# Autodesk Inventor assembly: Turtle3
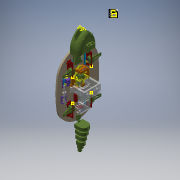
[picture p0: Inventor's stored thumbnail of the model, 180x180]
Saved by Autodesk Inventor 2018 (Build 220112000, 112)
## iProperties
Created: 2018-05-19
Part Number: Turtle3
Document SubType Name: Assembly
Designer: reide
Author: reide
## Documents named in this file (69)
- C:\Users\reide\OneDrive\Documents\Inventor\TSA\2018\Animatronics\Tortoise\Turtle3.iam
- C:\Users\reide\OneDrive\Documents\Inventor\TSA\2018\Animatronics\Tortoise\Frame\Frame - Copy.ipt
- C:\Users\reide\OneDrive\Documents\Inventor\TSA\2018\Animatronics\Tortoise\Rack.ipt
- C:\Users\reide\OneDrive\Documents\Inventor\TSA\2018\Animatronics\Tortoise\arms\Supporter.ipt
- C:\Users\reide\OneDrive\Documents\Inventor\TSA\2018\Animatronics\Tortoise\arms\GuideArm.ipt
- C:\Users\reide\OneDrive\Documents\Inventor\TSA\2018\Animatronics\Tortoise\arms\GuideArmConnector.ipt
- C:\Users\reide\OneDrive\Documents\Inventor\TSA\2018\Animatronics\Tortoise\arms\GuideArmConnectorLimitSwitch.ipt
- C:\Users\reide\OneDrive\Documents\Inventor\TSA\2018\Animatronics\Tortoise\arms\newShoulder_MIR.ipt
- C:\Users\reide\OneDrive\Documents\Inventor\TSA\2018\Animatronics\Tortoise\arms\straightBar_MIR.ipt
- C:\Users\reide\OneDrive\Documents\Inventor\TSA\2018\Animatronics\Tortoise\arms\AngleArm_MIR.ipt
- C:\Users\reide\OneDrive\Documents\Inventor\TSA\2018\Animatronics\Tortoise\arms\bottomARM_MIR.ipt
- C:\Users\reide\OneDrive\Documents\Inventor\TSA\2018\Animatronics\Tortoise\Mock Parts\servo (2)_MIR.ipt
- C:\Users\reide\OneDrive\Documents\Inventor\TSA\2018\Animatronics\Tortoise\Pinion final_MIR.ipt
- C:\Users\reide\OneDrive\Documents\Inventor\TSA\2018\Animatronics\Tortoise\arms\newShoulder.ipt
- C:\Users\reide\OneDrive\Documents\Inventor\TSA\2018\Animatronics\Tortoise\arms\straightBar.ipt
- C:\Users\reide\OneDrive\Documents\Inventor\TSA\2018\Animatronics\Tortoise\arms\AngleArm.ipt
- C:\Users\reide\OneDrive\Documents\Inventor\TSA\2018\Animatronics\Tortoise\arms\bottomARM.ipt
- C:\Users\reide\OneDrive\Documents\Inventor\TSA\2018\Animatronics\Tortoise\Mock Parts\servo (2).ipt
- C:\Users\reide\OneDrive\Documents\Inventor\TSA\2018\Animatronics\Tortoise\Pinion final.ipt
- C:\Users\reide\OneDrive\Documents\Inventor\TSA\2018\Animatronics\Tortoise\Head\HeadBasePt1.iam
- C:\Users\reide\OneDrive\Documents\Inventor\TSA\2018\Animatronics\Tortoise\Head\HeadBasePt2.iam
- C:\Users\reide\OneDrive\Documents\Inventor\TSA\2018\Animatronics\Tortoise\Head\HeadBottom1.ipt
- C:\Users\reide\OneDrive\Documents\Inventor\TSA\2018\Animatronics\Tortoise\Head\SyringeAttachment.ipt
- C:\Users\reide\OneDrive\Documents\Inventor\TSA\2018\Animatronics\Tortoise\Syringe3mL\SyringeBody.ipt
- C:\Users\reide\OneDrive\Documents\Inventor\TSA\2018\Animatronics\Tortoise\Syringe3mL\SyringEnd.ipt
- C:\Users\reide\OneDrive\Documents\Inventor\TSA\2018\Animatronics\Tortoise\Head\HeadBottom.ipt
- C:\Users\reide\OneDrive\Documents\Inventor\TSA\2018\Animatronics\Tortoise\Head\HeadLever.ipt
- C:\Users\reide\OneDrive\Documents\Inventor\TSA\2018\Animatronics\Tortoise\Head\FlexHinge.ipt
- C:\Users\reide\OneDrive\Documents\Inventor\TSA\2018\Animatronics\Tortoise\Head\HeadTop.ipt
- C:\Users\reide\OneDrive\Documents\Inventor\TSA\2018\Animatronics\Tortoise\Head\Face.ipt
- C:\Users\reide\OneDrive\Documents\Inventor\TSA\2018\Animatronics\Tortoise\Head\Eyes.ipt
- C:\Users\reide\OneDrive\Documents\Inventor\TSA\2018\Animatronics\Tortoise\Head\SensorMount.ipt
- C:\Users\reide\OneDrive\Documents\Inventor\TSA\2018\Animatronics\Tortoise\Wheels\smallergear.ipt
- C:\Users\reide\OneDrive\Documents\Inventor\TSA\2018\Animatronics\Tortoise\Clamps\SteerServoClamp.ipt
- C:\Users\reide\OneDrive\Documents\Inventor\TSA\2018\Animatronics\Tortoise\Wheels\steer_servo_mount1.ipt
- C:\Users\reide\OneDrive\Documents\Inventor\TSA\2018\Animatronics\Tortoise\Wheels\steer_servo_mount2.ipt
- C:\Users\reide\OneDrive\Documents\Inventor\TSA\2018\Animatronics\Tortoise\Wheels\wheelframe2NEW.ipt
- C:\Users\reide\OneDrive\Documents\Inventor\TSA\2018\Animatronics\Tortoise\Wheels\wheelframe.ipt
- C:\Users\reide\OneDrive\Documents\Inventor\TSA\2018\Animatronics\Tortoise\Wheels\wheel gear.ipt
- C:\Users\reide\OneDrive\Documents\Inventor\TSA\2018\Animatronics\Tortoise\Wheels\correct_wheel.ipt
- C:\Users\reide\OneDrive\Documents\Inventor\TSA\2018\Animatronics\Tortoise\Wheels\holder_gear_mount1.ipt
- C:\Users\reide\OneDrive\Documents\Inventor\TSA\2018\Animatronics\Tortoise\Wheels\holder_gear_mount2.ipt
- C:\Users\reide\OneDrive\Documents\Inventor\TSA\2018\Animatronics\Tortoise\Wheels\BackWheelMount.ipt
- C:\Users\reide\OneDrive\Documents\Inventor\TSA\2018\Animatronics\Tortoise\Wheels\BackWheelServoClasp.ipt
- C:\Users\reide\OneDrive\Documents\Inventor\TSA\2018\Animatronics\Tortoise\Wheels\Backwheel.ipt
- C:\Users\reide\OneDrive\Documents\Inventor\TSA\2018\Animatronics\Tortoise\Tail\Tail_Servo_Mount.ipt
- C:\Users\reide\OneDrive\Documents\Inventor\TSA\2018\Animatronics\Tortoise\Tail\Tail_Mount.ipt
- C:\Users\reide\OneDrive\Documents\Inventor\TSA\2018\Animatronics\Tortoise\Tail\Tail3.ipt
- C:\Users\reide\OneDrive\Documents\Inventor\TSA\2018\Animatronics\Tortoise\Tail\Tail4.ipt
- C:\Users\reide\OneDrive\Documents\Inventor\TSA\2018\Animatronics\Tortoise\Tail\Tail5.ipt
- C:\Users\reide\OneDrive\Documents\Inventor\TSA\2018\Animatronics\Tortoise\Tail\Tail6.ipt
- C:\Users\reide\OneDrive\Documents\Inventor\TSA\2018\Animatronics\Tortoise\Frame\TablePt1.ipt
- C:\Users\reide\OneDrive\Documents\Inventor\TSA\2018\Animatronics\Tortoise\Frame\TablePt2.ipt
- C:\Users\reide\OneDrive\Documents\Inventor\TSA\2018\Animatronics\Tortoise\Frame\TableLeg.ipt
- C:\Users\reide\OneDrive\Documents\Inventor\TSA\2018\Animatronics\Tortoise\Frame\ButtonMountLegs.ipt
- C:\Users\reide\OneDrive\Documents\Inventor\TSA\2018\Animatronics\Tortoise\Frame\ButtonMountCarrier.ipt
- C:\Users\reide\OneDrive\Documents\Inventor\TSA\2018\Animatronics\Tortoise\Frame\ButtonMount.ipt
- C:\Users\reide\OneDrive\Documents\Inventor\TSA\2018\Animatronics\Tortoise\Head\HeadOpenRack.ipt
- C:\Users\reide\OneDrive\Documents\Inventor\TSA\2018\Animatronics\Tortoise\Frame\SyringeMotorBase_MIR.ipt
- C:\Users\reide\OneDrive\Documents\Inventor\TSA\2018\Animatronics\Tortoise\Clamps\SyringeServoBaseClamp_MIR.ipt
- C:\Users\reide\OneDrive\Documents\Inventor\TSA\2018\Animatronics\Tortoise\Frame\BaseSyringeRackWall.ipt
- C:\Users\reide\OneDrive\Documents\Inventor\TSA\2018\Animatronics\Tortoise\Clamps\SyringeBaseSlotters.ipt
- C:\Users\reide\OneDrive\Documents\Inventor\TSA\2018\Animatronics\Tortoise\Head\SyringeHeadLeverAttachment.ipt
- C:\Users\reide\OneDrive\Documents\Inventor\TSA\2018\Animatronics\Tortoise\Head\LeverArm.ipt
- C:\Users\reide\OneDrive\Documents\Inventor\TSA\2018\Animatronics\Tortoise\Head\HeadLeverAssemblyAttacher.ipt
- C:\Users\reide\OneDrive\Documents\Inventor\TSA\2018\Animatronics\Tortoise\Frame\ThumbScrew.ipt
- C:\Users\reide\OneDrive\Documents\Inventor\TSA\2018\Animatronics\Tortoise\Clamps\SyringeServoClamp.ipt
- C:\Users\reide\OneDrive\Documents\Inventor\TSA\2018\Animatronics\Tortoise\Frame\ButtonLockerV2.ipt
- C:\Users\reide\OneDrive\Documents\Inventor\TSA\2018\Animatronics\Tortoise\Frame\FrameRim.ipt
## Components (131 placed, 68 different names)
1. Frame - Copy:1 — Mate:17, Mate:18, Mate:19, Mate:20, Mate:21, Mate:22, Mate:23, Mate:24, Mate:25, Mate:26, Mate:27, Mate:28, Mate:29, Mate:30, Mate:31, Mate:32, Mate:33, Mate:34, Mate:35, Mate:36, Mate:37, Mate:38, Mate:39, Mate:40, Mate:41, Mate:88, Mate:89, Mate:90, Mate:144, Mate:145, Mate:157, Mate:158, Mate:161, Mate:162, Mate:167, Mate:168, Mate:169, Mate:175, Mate:176, Mate:177, Mate:178, Mate:179, Mate:180, Mate:181, Mate:182, Mate:183, Mate:184, Mate:185, Mate:186, Mate:187, Mate:203, Mate:204, Mate:205, Mate:206, Mate:207, Mate:208, Mate:209, Mate:210, Mate:241, Mate:242, Mate:243, Mate:244, Mate:245, Flush:106, Mate:246, Mate:247, Flush:107, Mate:248, Mate:249, Mate:250, Mate:254, Flush:111, Mate:295, Mate:296, Flush:114
2. Rack:1 — Flush:6, Flush:25, Flush:26, Flush:27, Mate:22, Mate:23
3. Supporter:1 — Flush:5, Flush:6, Mate:17, Mate:18, Mate:19, Mate:51, Angle:9
4. GuideArm:1 — Mate:52
5. GuideArmConnector:1 — Mate:21
6. GuideArmConnectorLimitSwitch:1 — Flush:5, Mate:20
7. Rack:2 — Mate:28, Mate:29
8. Supporter:2 — Flush:25, Mate:24, Mate:25, Mate:80
9. GuideArm:2 — Mate:81
10. GuideArmConnector:2 — Mate:27
11. GuideArmConnectorLimitSwitch:2 — Mate:26
12. Rack:3 — Mate:40, Mate:41
13. Supporter:3 — Flush:27, Mate:36, Mate:37, Mate:85
14. GuideArm:3 — Mate:84
15. GuideArmConnector:3 — Mate:38
16. GuideArmConnectorLimitSwitch:3 — Mate:39
17. Rack:4 — Mate:34, Mate:35
18. Supporter:4 — Flush:26, Mate:30, Mate:31, Mate:83
19. GuideArm:4 — Mate:82
20. GuideArmConnector:4 — Mate:32
21. GuideArmConnectorLimitSwitch:4 — Mate:33
22. newShoulder_MIR:1 — Mate:50, Mate:51, Mate:52
23. straightBar_MIR:1
24. AngleArm_MIR:1 — Angle:8
25. bottomARM_MIR:1
26. servo (2)_MIR:1 — Mate:50
27. Pinion final_MIR:1
28. newShoulder_MIR:2 — Mate:84, Mate:85
29. straightBar_MIR:2
30. AngleArm_MIR:2
31. bottomARM_MIR:2
32. servo (2)_MIR:2
33. Pinion final_MIR:2
34. newShoulder:1 — Mate:70, Mate:80, Mate:81
35. straightBar:1
36. AngleArm:1
37. bottomARM:1
38. servo (2):1 — Mate:70
39. Pinion final:1
40. newShoulder:2 — Mate:82, Mate:83
41. straightBar:2
42. AngleArm:2
43. bottomARM:2
44. servo (2):2
45. Pinion final:2
46. HeadBasePt1:1 [sub-assembly] — Mate:86, Flush:48, Mate:87, Mate:89, Mate:90, Mate:127, Mate:128, Angle:2, Angle:3
47. HeadBasePt2:1 [sub-assembly] — Mate:86, Flush:48, Mate:87, Mate:88
48. servo (2):3 — Mate:131, Mate:132
49. HeadBottom1:1 — Mate:107, Mate:127, Mate:128, Angle:2, Flush:108, Mate:271, Mate:272
50. SyringeAttachment:1 — Angle:1
51. SyringeAttachment:2
52. servo (2):4 — Mate:129, Mate:130
53. SyringeBody:1 — Angle:1, Mate:107
54. SyringEnd:1 — Mate:261, Mate:262
55. HeadLever:1 — Mate:263, Mate:267, Mate:270, Mate:282, Mate:283, Mate:285
56. FlexHinge:1 — Mate:274, Mate:276, Angle:10
57. HeadTop:1 — Mate:119, Mate:263, Flush:110, Mate:284, Mate:285
58. Face:1 — Mate:119, Mate:120, Mate:298, Mate:299
59. FlexHinge:2 — Mate:273, Mate:275, Angle:9
60. Eyes:1 — Mate:120
61. Eyes:2
62. Pinion final:3 — Mate:129, Mate:130
63. Pinion final:4 — Mate:131, Mate:132
64. servo (2):5 — Mate:136, Mate:137, Mate:138, Mate:139, Mate:140
65. smallergear:1 — Mate:139, Mate:140
66. SteerServoClamp:1 — Mate:141, Mate:142, Mate:143
67. steer_servo_mount1:1 — Mate:134, Mate:135, Flush:54, Flush:55, Flush:56, Flush:57, Mate:136, Mate:137, Mate:138, Mate:141, Mate:142, Mate:143, Angle:3, Angle:4
68. steer_servo_mount2:1 — Mate:134, Flush:56, Flush:57, Mate:144, Mate:145
69. steer_servo_mount2:2 — Mate:135, Flush:54, Flush:55, Angle:5
70. wheelframe2NEW:1 — Mate:158
71. wheelframe:1 — Mate:153, Mate:154, Mate:155, Mate:157
72. wheel gear:1 — Flush:58, Mate:156
73. correct_wheel:1 — Flush:58
74. servo (2):7 — Mate:153, Mate:154, Mate:155, Mate:156
75. smallergear:2 — Flush:64, Mate:160
76. holder_gear_mount1:1 — Mate:159, Flush:60, Flush:61, Flush:62, Flush:63, Flush:64, Mate:160, Angle:4
77. holder_gear_mount2:1 — Flush:59, Mate:159, Flush:60, Flush:61, Mate:161, Mate:162
78. holder_gear_mount2:2 — Flush:59, Flush:62, Flush:63, Angle:6
79. smallergear:3
80. holder_gear_mount1:2
81. holder_gear_mount2:3 — Flush:77, Mate:167, Mate:169, Angle:6
82. holder_gear_mount2:4
83. smallergear:4
84. holder_gear_mount1:3
85. holder_gear_mount2:5 — Flush:77, Mate:168, Angle:5
86. holder_gear_mount2:6 — Angle:7
87. BackWheelMount:1 — Mate:178, Mate:179, Mate:180
88. BackWheelServoClasp:1 — Flush:79, Mate:175, Mate:176, Mate:177
89. Backwheel:1 — Mate:181
90. Tail_Servo_Mount:1 — Mate:182, Mate:183, Mate:184
91. servo (2):8 — Flush:79
92. servo (2):9
93. Tail_Mount:1 — Mate:185, Mate:186, Mate:187, Mate:188, Mate:189
94. Tail3:1 — Mate:188, Mate:189, Mate:190, Mate:191
95. Tail4:1 — Mate:190, Mate:191, Mate:192, Mate:193
96. Tail5:1 — Mate:192, Mate:193, Mate:194, Mate:195
97. Tail6:1 — Mate:194, Mate:195
98. TablePt1:1 — Mate:196, Flush:80, Flush:86, Mate:199, Mate:201, Mate:202, Flush:88, Mate:203
99. TablePt2:1 — Mate:196, Flush:80, Mate:198, Flush:81, Flush:82, Flush:87, Mate:200, Flush:88, Angle:7, Mate:286, Flush:112, Flush:113
100. TableLeg:1 — Mate:198, Flush:81, Flush:82, Flush:85
101. TableLeg:2 — Flush:83, Mate:201, Mate:202, Mate:204
102. TableLeg:3 — Flush:83, Flush:84, Flush:87, Mate:200
103. TableLeg:4 — Flush:84, Flush:85, Flush:86, Mate:199
104. ButtonMountLegs:1 — Mate:205, Mate:206, Mate:207, Mate:211, Angle:12
105. ButtonMountLegs:2 — Mate:208, Mate:209, Mate:210, Flush:90, Flush:91
106. ButtonMount:1 — Flush:90, Flush:91, Mate:211, Mate:287, Mate:288, Angle:11
107. SyringeBody:3 — Mate:245, Mate:297
108. SyringeAttachment:5 — Mate:247
109. SyringeAttachment:6 — Mate:246
110. servo (2)_MIR:4 — Mate:239, Flush:105, Mate:240
111. Pinion final:6
112. SyringeMotorBase_MIR:1 — Flush:103, Flush:104, Mate:238, Mate:239, Flush:105, Mate:240, Mate:241, Mate:242, Mate:243, Mate:244
113. SyringeServoBaseClamp_MIR:1 — Flush:103, Flush:104, Mate:238
114. BaseSyringeRackWall:1 — Flush:106, Mate:253, Mate:295, Mate:296
115. SyringeBaseSlotters:1 — Flush:107
116. SyringeBaseSlotters:2 — Mate:248, Mate:249, Mate:250
117. HeadOpenRack:3 — Mate:253, Mate:254
118. SyringEnd:4 — Mate:297
119. SyringeHeadLeverAttachment:1 — Mate:261, Mate:262, Angle:8, Mate:265, Mate:266, Mate:268, Mate:269
120. LeverArm:2 — Mate:265, Mate:266, Mate:267
121. LeverArm:3 — Mate:268, Mate:269, Mate:270
122. HeadLeverAssemblyAttacher:1 — Mate:277, Mate:278, Mate:279, Flush:109, Mate:282, Mate:283
123. HeadBottom:2 — Flush:108, Mate:271, Mate:272, Mate:273, Mate:274, Mate:275, Mate:276, Angle:10, Mate:277, Mate:278, Mate:279, Mate:280, Mate:281, Flush:110, Mate:284, Angle:14
124. HeadLeverAssemblyAttacher:2 — Mate:280, Flush:109, Mate:281
125. ThumbScrew:1 — Flush:111
126. SyringeServoClamp:1 — Mate:286, Flush:112, Flush:113
127. ButtonMountCarrier:2 — Mate:287, Mate:288, Angle:11, Mate:292, Angle:13
128. ButtonLockerV2:2 — Mate:292, Angle:12
129. ButtonLockerV2:3 — Angle:13
130. FrameRim:1 — Flush:114
131. SensorMount:2 — Mate:298, Angle:14, Mate:299
## Relationships (361: Mate 249, Flush 98, Angle 14)
- [Flush]: Rack:1 ↔ Supporter:1
- [Mate]: GuideArm:1 ↔ GuideArmConnector:1
- [Mate]: GuideArm:1 ↔ GuideArmConnector:1
- [Flush]: GuideArm:1 ↔ GuideArmConnector:1
- [Flush]: GuideArmConnector:1 ↔ GuideArmConnectorLimitSwitch:1
- [Mate]: GuideArm:1 ↔ GuideArmConnectorLimitSwitch:1
- [Flush]: GuideArm:1 ↔ GuideArmConnectorLimitSwitch:1
- [Mate]: GuideArm:1 ↔ GuideArmConnectorLimitSwitch:1
- Flush:5: Supporter:1 ↔ GuideArmConnectorLimitSwitch:1
- Flush:6: Rack:1 ↔ Supporter:1
- [Flush]: Rack:2 ↔ Supporter:2
- [Mate]: GuideArm:2 ↔ GuideArmConnector:2
- [Mate]: GuideArm:2 ↔ GuideArmConnector:2
- [Flush]: GuideArm:2 ↔ GuideArmConnector:2
- [Flush]: GuideArmConnector:2 ↔ GuideArmConnectorLimitSwitch:2
- [Mate]: GuideArm:2 ↔ GuideArmConnectorLimitSwitch:2
- [Flush]: GuideArm:2 ↔ GuideArmConnectorLimitSwitch:2
- [Mate]: GuideArm:2 ↔ GuideArmConnectorLimitSwitch:2
- [Flush]: Supporter:2 ↔ GuideArmConnectorLimitSwitch:2
- [Flush]: Rack:2 ↔ Supporter:2
- [Flush]: Rack:3 ↔ Supporter:3
- [Mate]: GuideArm:3 ↔ GuideArmConnector:3
- [Mate]: GuideArm:3 ↔ GuideArmConnector:3
- [Flush]: GuideArm:3 ↔ GuideArmConnector:3
- [Flush]: GuideArmConnector:3 ↔ GuideArmConnectorLimitSwitch:3
- [Mate]: GuideArm:3 ↔ GuideArmConnectorLimitSwitch:3
- [Flush]: GuideArm:3 ↔ GuideArmConnectorLimitSwitch:3
- [Mate]: GuideArm:3 ↔ GuideArmConnectorLimitSwitch:3
- [Flush]: Supporter:3 ↔ GuideArmConnectorLimitSwitch:3
- [Flush]: Rack:3 ↔ Supporter:3
- [Flush]: Rack:4 ↔ Supporter:4
- [Mate]: GuideArm:4 ↔ GuideArmConnector:4
- [Mate]: GuideArm:4 ↔ GuideArmConnector:4
- [Flush]: GuideArm:4 ↔ GuideArmConnector:4
- [Flush]: GuideArmConnector:4 ↔ GuideArmConnectorLimitSwitch:4
- [Mate]: GuideArm:4 ↔ GuideArmConnectorLimitSwitch:4
- [Flush]: GuideArm:4 ↔ GuideArmConnectorLimitSwitch:4
- [Mate]: GuideArm:4 ↔ GuideArmConnectorLimitSwitch:4
- [Flush]: Supporter:4 ↔ GuideArmConnectorLimitSwitch:4
- [Flush]: Rack:4 ↔ Supporter:4
- Mate:17: Frame - Copy:1 ↔ Supporter:1
- Flush:25: Rack:1 ↔ Supporter:2
- Flush:26: Rack:1 ↔ Supporter:4
- Flush:27: Rack:1 ↔ Supporter:3
- Mate:18: Frame - Copy:1 ↔ Supporter:1
- Mate:19: Frame - Copy:1 ↔ Supporter:1
- Mate:20: Frame - Copy:1 ↔ GuideArmConnectorLimitSwitch:1
- Mate:21: Frame - Copy:1 ↔ GuideArmConnector:1
- Mate:22: Frame - Copy:1 ↔ Rack:1
- Mate:23: Frame - Copy:1 ↔ Rack:1
- Mate:24: Frame - Copy:1 ↔ Supporter:2
- Mate:25: Frame - Copy:1 ↔ Supporter:2
- Mate:26: Frame - Copy:1 ↔ GuideArmConnectorLimitSwitch:2
- Mate:27: Frame - Copy:1 ↔ GuideArmConnector:2
- Mate:28: Frame - Copy:1 ↔ Rack:2
- Mate:29: Frame - Copy:1 ↔ Rack:2
- Mate:30: Frame - Copy:1 ↔ Supporter:4
- Mate:31: Frame - Copy:1 ↔ Supporter:4
- Mate:32: Frame - Copy:1 ↔ GuideArmConnector:4
- Mate:33: Frame - Copy:1 ↔ GuideArmConnectorLimitSwitch:4
- Mate:34: Frame - Copy:1 ↔ Rack:4
- Mate:35: Frame - Copy:1 ↔ Rack:4
- Mate:36: Frame - Copy:1 ↔ Supporter:3
- Mate:37: Frame - Copy:1 ↔ Supporter:3
- Mate:38: Frame - Copy:1 ↔ GuideArmConnector:3
- Mate:39: Frame - Copy:1 ↔ GuideArmConnectorLimitSwitch:3
- Mate:40: Frame - Copy:1 ↔ Rack:3
- Mate:41: Frame - Copy:1 ↔ Rack:3
- [Mate]: newShoulder_MIR:1 ↔ straightBar_MIR:1
- [Mate]: newShoulder_MIR:1 ↔ straightBar_MIR:1
- [Flush]: newShoulder_MIR:1 ↔ straightBar_MIR:1
- [Mate]: newShoulder_MIR:1 ↔ AngleArm_MIR:1
- [Mate]: newShoulder_MIR:1 ↔ AngleArm_MIR:1
- [Flush]: newShoulder_MIR:1 ↔ AngleArm_MIR:1
- [Flush]: newShoulder_MIR:1 ↔ bottomARM_MIR:1
- [Flush]: newShoulder_MIR:1 ↔ bottomARM_MIR:1
- [Mate]: newShoulder_MIR:1 ↔ bottomARM_MIR:1
- [Flush]: newShoulder_MIR:1 ↔ servo (2)_MIR:1
- [Mate]: newShoulder_MIR:1 ↔ servo (2)_MIR:1
- [Mate]: servo (2)_MIR:1 ↔ Pinion final_MIR:1
- [Mate]: servo (2)_MIR:1 ↔ Pinion final_MIR:1
- Mate:50 (0.5 mm): newShoulder_MIR:1 ↔ servo (2)_MIR:1
- Mate:51: Supporter:1 ↔ newShoulder_MIR:1
- Mate:52 (0.125 mm): GuideArm:1 ↔ newShoulder_MIR:1
- [Mate]: newShoulder_MIR:2 ↔ straightBar_MIR:2
- [Mate]: newShoulder_MIR:2 ↔ straightBar_MIR:2
- [Flush]: newShoulder_MIR:2 ↔ straightBar_MIR:2
- [Mate]: newShoulder_MIR:2 ↔ AngleArm_MIR:2
- [Mate]: newShoulder_MIR:2 ↔ AngleArm_MIR:2
- [Flush]: newShoulder_MIR:2 ↔ AngleArm_MIR:2
- [Flush]: newShoulder_MIR:2 ↔ bottomARM_MIR:2
- [Flush]: newShoulder_MIR:2 ↔ bottomARM_MIR:2
- [Mate]: newShoulder_MIR:2 ↔ bottomARM_MIR:2
- [Flush]: newShoulder_MIR:2 ↔ servo (2)_MIR:2
- [Mate]: newShoulder_MIR:2 ↔ servo (2)_MIR:2
- [Mate]: servo (2)_MIR:2 ↔ Pinion final_MIR:2
- [Mate]: servo (2)_MIR:2 ↔ Pinion final_MIR:2
- [Mate] (0.5 mm): newShoulder_MIR:2 ↔ servo (2)_MIR:2
- [Flush]: newShoulder:1 ↔ AngleArm:1
- [Mate]: newShoulder:1 ↔ AngleArm:1
- [Mate]: newShoulder:1 ↔ AngleArm:1
- [Flush]: newShoulder:1 ↔ straightBar:1
- [Mate]: newShoulder:1 ↔ straightBar:1
- [Mate]: newShoulder:1 ↔ straightBar:1
- [Mate]: newShoulder:1 ↔ bottomARM:1
- [Flush]: newShoulder:1 ↔ bottomARM:1
- [Flush]: newShoulder:1 ↔ bottomARM:1
- [Mate]: newShoulder:1 ↔ servo (2):1
- [Flush]: newShoulder:1 ↔ servo (2):1
- [Mate]: servo (2):1 ↔ Pinion final:1
- [Mate]: servo (2):1 ↔ Pinion final:1
- Mate:70 (0.5 mm): newShoulder:1 ↔ servo (2):1
- [Flush]: newShoulder:2 ↔ AngleArm:2
- [Mate]: newShoulder:2 ↔ AngleArm:2
- [Mate]: newShoulder:2 ↔ AngleArm:2
- [Flush]: newShoulder:2 ↔ straightBar:2
- [Mate]: newShoulder:2 ↔ straightBar:2
- [Mate]: newShoulder:2 ↔ straightBar:2
- [Mate]: newShoulder:2 ↔ bottomARM:2
- [Flush]: newShoulder:2 ↔ bottomARM:2
- [Flush]: newShoulder:2 ↔ bottomARM:2
- [Mate]: newShoulder:2 ↔ servo (2):2
- [Flush]: newShoulder:2 ↔ servo (2):2
- [Mate]: servo (2):2 ↔ Pinion final:2
- [Mate]: servo (2):2 ↔ Pinion final:2
- [Mate] (0.5 mm): newShoulder:2 ↔ servo (2):2
- Mate:80: Supporter:2 ↔ newShoulder:1
- Mate:81 (0.125 mm): GuideArm:2 ↔ newShoulder:1
- Mate:82 (0.125 mm): GuideArm:4 ↔ newShoulder:2
- Mate:83: Supporter:4 ↔ newShoulder:2
- Mate:84 (0.125 mm): GuideArm:3 ↔ newShoulder_MIR:2
- Mate:85: Supporter:3 ↔ newShoulder_MIR:2
- Mate:86 (0.25 mm): HeadBasePt1:1 ↔ HeadBasePt2:1
- Flush:48: HeadBasePt1:1 ↔ HeadBasePt2:1
- Mate:87: HeadBasePt1:1 ↔ HeadBasePt2:1
- Mate:88: Frame - Copy:1 ↔ HeadBasePt2:1
- Mate:89: Frame - Copy:1 ↔ HeadBasePt1:1
- Mate:90: Frame - Copy:1 ↔ HeadBasePt1:1
- [Mate]: HeadBottom1:1 ↔ servo (2):4
- [Mate] (0.25 mm): HeadBottom1:1 ↔ servo (2):4
- [Mate] (0.25 mm): HeadBottom1:1 ↔ servo (2):4
- [Mate]: servo (2):3 ↔ HeadBottom1:1
- [Mate] (0.25 mm): servo (2):3 ↔ HeadBottom1:1
- [Mate] (0.25 mm): servo (2):3 ↔ HeadBottom1:1
- [Mate] (0.25 mm): HeadBottom1:1 ↔ SyringeAttachment:2
- [Mate] (0.25 mm): HeadBottom1:1 ↔ SyringeAttachment:1
- [Mate]: HeadBottom1:1 ↔ SyringeAttachment:2
- [Mate] (0.25 mm): HeadBottom1:1 ↔ SyringeAttachment:2
- [Mate] (0.25 mm): HeadBottom1:1 ↔ SyringeAttachment:2
- [Mate]: HeadBottom1:1 ↔ SyringeAttachment:1
- [Mate] (0.25 mm): HeadBottom1:1 ↔ SyringeAttachment:1
- [Mate] (0.25 mm): HeadBottom1:1 ↔ SyringeAttachment:1
- [Mate]: SyringeAttachment:2 ↔ SyringeBody:1
- [Mate]: SyringeBody:1 ↔ SyringEnd:1
- Angle:1 (0 deg): SyringeAttachment:1 ↔ SyringeBody:1
- Mate:107: HeadBottom1:1 ↔ SyringeBody:1
- [Mate]: HeadTop:1 ↔ Face:1
- [Mate]: HeadTop:1 ↔ Face:1
- [Flush]: Face:1 ↔ Eyes:1
- [Mate]: Face:1 ↔ Eyes:2
- [Mate]: Face:1 ↔ Eyes:2
- Mate:119: HeadTop:1 ↔ Face:1
- Mate:120: Face:1 ↔ Eyes:1
- Mate:127: HeadBasePt1:1 ↔ HeadBottom1:1
- Mate:128 (1.75 mm): HeadBasePt1:1 ↔ HeadBottom1:1
- Angle:2 (0 deg): HeadBasePt1:1 ↔ HeadBottom1:1
- Mate:129: servo (2):4 ↔ Pinion final:3
- Mate:130: servo (2):4 ↔ Pinion final:3
- Mate:131: servo (2):3 ↔ Pinion final:4
- Mate:132: servo (2):3 ↔ Pinion final:4
- [Mate]: servo (2):5 ↔ smallergear:1
- Mate:134: steer_servo_mount1:1 ↔ steer_servo_mount2:1
- Mate:135: steer_servo_mount1:1 ↔ steer_servo_mount2:2
- Flush:54: steer_servo_mount1:1 ↔ steer_servo_mount2:2
- Flush:55: steer_servo_mount1:1 ↔ steer_servo_mount2:2
- Flush:56: steer_servo_mount1:1 ↔ steer_servo_mount2:1
- Flush:57: steer_servo_mount1:1 ↔ steer_servo_mount2:1
- Mate:136: servo (2):5 ↔ steer_servo_mount1:1
- Mate:137: servo (2):5 ↔ steer_servo_mount1:1
- Mate:138 (0.5 mm): servo (2):5 ↔ steer_servo_mount1:1
- Mate:139: servo (2):5 ↔ smallergear:1
- Mate:140: servo (2):5 ↔ smallergear:1
- Mate:141: SteerServoClamp:1 ↔ steer_servo_mount1:1
- Mate:142: SteerServoClamp:1 ↔ steer_servo_mount1:1
- Mate:143: SteerServoClamp:1 ↔ steer_servo_mount1:1
- Mate:144: Frame - Copy:1 ↔ steer_servo_mount2:1
- Mate:145 (1.5 mm): Frame - Copy:1 ↔ steer_servo_mount2:1
- Angle:3 (0 deg): HeadBasePt1:1 ↔ steer_servo_mount1:1
- [Mate]: wheelframe2NEW:1 ↔ wheelframe:1
- [Mate]: wheelframe2NEW:1 ↔ wheelframe:1
- [Mate]: wheelframe2NEW:1 ↔ correct_wheel:1
- [Mate]: wheelframe2NEW:1 ↔ wheel gear:1
- [Mate]: wheelframe2NEW:1 ↔ wheelframe:1
- Mate:153: wheelframe:1 ↔ servo (2):7
- Mate:154: wheelframe:1 ↔ servo (2):7
- Mate:155: wheelframe:1 ↔ servo (2):7
- Flush:58: wheel gear:1 ↔ correct_wheel:1
- Mate:156: wheel gear:1 ↔ servo (2):7
- Mate:157: Frame - Copy:1 ↔ wheelframe:1
- Mate:158: Frame - Copy:1 ↔ wheelframe2NEW:1
- Flush:59: holder_gear_mount2:1 ↔ holder_gear_mount2:2
- Mate:159: holder_gear_mount1:1 ↔ holder_gear_mount2:1
- Flush:60: holder_gear_mount1:1 ↔ holder_gear_mount2:1
- Flush:61: holder_gear_mount1:1 ↔ holder_gear_mount2:1
- Flush:62: holder_gear_mount1:1 ↔ holder_gear_mount2:2
- Flush:63: holder_gear_mount1:1 ↔ holder_gear_mount2:2
- Flush:64: smallergear:2 ↔ holder_gear_mount1:1
- Mate:160: smallergear:2 ↔ holder_gear_mount1:1
- Mate:161: Frame - Copy:1 ↔ holder_gear_mount2:1
- Mate:162 (1.5 mm): Frame - Copy:1 ↔ holder_gear_mount2:1
- Angle:4 (0 deg): steer_servo_mount1:1 ↔ holder_gear_mount1:1
- [Flush]: holder_gear_mount2:3 ↔ holder_gear_mount2:4
- [Mate]: holder_gear_mount1:2 ↔ holder_gear_mount2:3
- [Flush]: holder_gear_mount1:2 ↔ holder_gear_mount2:3
- [Flush]: holder_gear_mount1:2 ↔ holder_gear_mount2:3
- [Flush]: holder_gear_mount1:2 ↔ holder_gear_mount2:4
- [Flush]: holder_gear_mount1:2 ↔ holder_gear_mount2:4
- [Flush]: smallergear:3 ↔ holder_gear_mount1:2
- [Mate]: smallergear:3 ↔ holder_gear_mount1:2
- [Flush]: holder_gear_mount2:5 ↔ holder_gear_mount2:6
- [Mate]: holder_gear_mount1:3 ↔ holder_gear_mount2:5
- [Flush]: holder_gear_mount1:3 ↔ holder_gear_mount2:5
- [Flush]: holder_gear_mount1:3 ↔ holder_gear_mount2:5
- [Flush]: holder_gear_mount1:3 ↔ holder_gear_mount2:6
- [Flush]: holder_gear_mount1:3 ↔ holder_gear_mount2:6
- [Flush]: smallergear:4 ↔ holder_gear_mount1:3
- [Mate]: smallergear:4 ↔ holder_gear_mount1:3
- Flush:77: holder_gear_mount2:3 ↔ holder_gear_mount2:5
- Mate:167: Frame - Copy:1 ↔ holder_gear_mount2:3
- Mate:168 (1.5 mm): Frame - Copy:1 ↔ holder_gear_mount2:5
- Angle:5 (0 deg): steer_servo_mount2:2 ↔ holder_gear_mount2:5
- Mate:169 (1.5 mm): Frame - Copy:1 ↔ holder_gear_mount2:3
- Angle:6 (0 deg): holder_gear_mount2:2 ↔ holder_gear_mount2:3
- [Mate]: BackWheelMount:1 ↔ Backwheel:1
- [Mate]: Tail_Servo_Mount:1 ↔ servo (2):9
- [Mate]: Tail_Servo_Mount:1 ↔ servo (2):9
- [Flush]: Tail_Servo_Mount:1 ↔ servo (2):9
- [Mate]: BackWheelServoClasp:1 ↔ servo (2):8
- [Mate] (1 mm): BackWheelServoClasp:1 ↔ servo (2):8
- Flush:79: BackWheelServoClasp:1 ↔ servo (2):8
- Mate:175: Frame - Copy:1 ↔ BackWheelServoClasp:1
- Mate:176: Frame - Copy:1 ↔ BackWheelServoClasp:1
- Mate:177: Frame - Copy:1 ↔ BackWheelServoClasp:1
- Mate:178: Frame - Copy:1 ↔ BackWheelMount:1
- Mate:179: Frame - Copy:1 ↔ BackWheelMount:1
- Mate:180: Frame - Copy:1 ↔ BackWheelMount:1
- Mate:181 (2.5 mm): Frame - Copy:1 ↔ Backwheel:1
- Mate:182: Frame - Copy:1 ↔ Tail_Servo_Mount:1
- Mate:183: Frame - Copy:1 ↔ Tail_Servo_Mount:1
- Mate:184: Frame - Copy:1 ↔ Tail_Servo_Mount:1
- Mate:185: Frame - Copy:1 ↔ Tail_Mount:1
- Mate:186: Frame - Copy:1 ↔ Tail_Mount:1
- Mate:187: Frame - Copy:1 ↔ Tail_Mount:1
- Mate:188: Tail_Mount:1 ↔ Tail3:1
- Mate:189: Tail_Mount:1 ↔ Tail3:1
- Mate:190: Tail3:1 ↔ Tail4:1
- Mate:191: Tail3:1 ↔ Tail4:1
- Mate:192: Tail4:1 ↔ Tail5:1
- Mate:193: Tail4:1 ↔ Tail5:1
- Mate:194: Tail5:1 ↔ Tail6:1
- Mate:195: Tail5:1 ↔ Tail6:1
- Mate:196: TablePt1:1 ↔ TablePt2:1
- Flush:80: TablePt1:1 ↔ TablePt2:1
- Mate:198: TablePt2:1 ↔ TableLeg:1
- Flush:81: TablePt2:1 ↔ TableLeg:1
- Flush:82: TablePt2:1 ↔ TableLeg:1
- Flush:83: TableLeg:2 ↔ TableLeg:3
- Flush:84: TableLeg:3 ↔ TableLeg:4
- Flush:85: TableLeg:1 ↔ TableLeg:4
- Flush:86: TablePt1:1 ↔ TableLeg:4
- Mate:199 (0.25 mm): TablePt1:1 ↔ TableLeg:4
- Flush:87: TablePt2:1 ↔ TableLeg:3
- Mate:200 (0.25 mm): TablePt2:1 ↔ TableLeg:3
- Mate:201: TablePt1:1 ↔ TableLeg:2
- Mate:202 (0.25 mm): TablePt1:1 ↔ TableLeg:2
- Flush:88: TablePt1:1 ↔ TablePt2:1
- Mate:203: Frame - Copy:1 ↔ TablePt1:1
- Mate:204: Frame - Copy:1 ↔ TableLeg:2
- Angle:7 (0 deg): holder_gear_mount2:6 ↔ TablePt2:1
- Mate:205: Frame - Copy:1 ↔ ButtonMountLegs:1
- Mate:206: Frame - Copy:1 ↔ ButtonMountLegs:1
- Mate:207: Frame - Copy:1 ↔ ButtonMountLegs:1
- Mate:208: Frame - Copy:1 ↔ ButtonMountLegs:2
- Mate:209: Frame - Copy:1 ↔ ButtonMountLegs:2
- Mate:210: Frame - Copy:1 ↔ ButtonMountLegs:2
- Flush:90: ButtonMountLegs:2 ↔ ButtonMount:1
- Flush:91: ButtonMountLegs:2 ↔ ButtonMount:1
- Mate:211: ButtonMountLegs:1 ↔ ButtonMount:1
- [Mate]: SyringeBody:3 ↔ SyringeAttachment:6
- [Mate]: SyringeBody:3 ↔ SyringeAttachment:5
- [Mate]: servo (2)_MIR:4 ↔ Pinion final:6
- [Mate]: servo (2)_MIR:4 ↔ Pinion final:6
- Flush:103: SyringeMotorBase_MIR:1 ↔ SyringeServoBaseClamp_MIR:1
- Flush:104: SyringeMotorBase_MIR:1 ↔ SyringeServoBaseClamp_MIR:1
- Mate:238: SyringeMotorBase_MIR:1 ↔ SyringeServoBaseClamp_MIR:1
- Mate:239: servo (2)_MIR:4 ↔ SyringeMotorBase_MIR:1
- Flush:105: servo (2)_MIR:4 ↔ SyringeMotorBase_MIR:1
- Mate:240 (0.25 mm): servo (2)_MIR:4 ↔ SyringeMotorBase_MIR:1
- Mate:241: Frame - Copy:1 ↔ SyringeMotorBase_MIR:1
- Mate:242: Frame - Copy:1 ↔ SyringeMotorBase_MIR:1
- Mate:243: Frame - Copy:1 ↔ SyringeMotorBase_MIR:1
- Mate:244: Frame - Copy:1 ↔ SyringeMotorBase_MIR:1
- Mate:245: Frame - Copy:1 ↔ SyringeBody:3
- Flush:106: Frame - Copy:1 ↔ BaseSyringeRackWall:1
- Mate:246: Frame - Copy:1 ↔ SyringeAttachment:6
- Mate:247: Frame - Copy:1 ↔ SyringeAttachment:5
- Flush:107: Frame - Copy:1 ↔ SyringeBaseSlotters:1
- Mate:248: Frame - Copy:1 ↔ SyringeBaseSlotters:2
- Mate:249: Frame - Copy:1 ↔ SyringeBaseSlotters:2
- Mate:250: Frame - Copy:1 ↔ SyringeBaseSlotters:2
- [Mate]: HeadOpenRack:3 ↔ SyringEnd:4
- [Mate]: HeadOpenRack:3 ↔ SyringEnd:4
- Mate:253 (0.5 mm): BaseSyringeRackWall:1 ↔ HeadOpenRack:3
- Mate:254: Frame - Copy:1 ↔ HeadOpenRack:3
- Mate:261: SyringEnd:1 ↔ SyringeHeadLeverAttachment:1
- Mate:262: SyringEnd:1 ↔ SyringeHeadLeverAttachment:1
- Angle:8 (0 deg): AngleArm_MIR:1 ↔ SyringeHeadLeverAttachment:1
- Mate:263: HeadLever:1 ↔ HeadTop:1
- Mate:265: SyringeHeadLeverAttachment:1 ↔ LeverArm:2
- Mate:266: SyringeHeadLeverAttachment:1 ↔ LeverArm:2
- Mate:267: HeadLever:1 ↔ LeverArm:2
- Mate:268: SyringeHeadLeverAttachment:1 ↔ LeverArm:3
- Mate:269: SyringeHeadLeverAttachment:1 ↔ LeverArm:3
- Mate:270: HeadLever:1 ↔ LeverArm:3
- Flush:108: HeadBottom1:1 ↔ HeadBottom:2
- Mate:271: HeadBottom1:1 ↔ HeadBottom:2
- Mate:272 (0.25 mm): HeadBottom1:1 ↔ HeadBottom:2
- Mate:273: FlexHinge:2 ↔ HeadBottom:2
- Mate:274: FlexHinge:1 ↔ HeadBottom:2
- Mate:275: FlexHinge:2 ↔ HeadBottom:2
- Mate:276: FlexHinge:1 ↔ HeadBottom:2
- Angle:9 (0 deg): Supporter:1 ↔ FlexHinge:2
- Angle:10 (0 deg): FlexHinge:1 ↔ HeadBottom:2
- Mate:277: HeadLeverAssemblyAttacher:1 ↔ HeadBottom:2
- Mate:278 (0.25 mm): HeadLeverAssemblyAttacher:1 ↔ HeadBottom:2
- Mate:279 (0.25 mm): HeadLeverAssemblyAttacher:1 ↔ HeadBottom:2
- Mate:280: HeadBottom:2 ↔ HeadLeverAssemblyAttacher:2
- Flush:109: HeadLeverAssemblyAttacher:1 ↔ HeadLeverAssemblyAttacher:2
- Mate:281 (0.25 mm): HeadBottom:2 ↔ HeadLeverAssemblyAttacher:2
- Mate:282: HeadLever:1 ↔ HeadLeverAssemblyAttacher:1
- Mate:283 (0.25 mm): HeadLever:1 ↔ HeadLeverAssemblyAttacher:1
- Flush:110: HeadTop:1 ↔ HeadBottom:2
- Mate:284: HeadTop:1 ↔ HeadBottom:2
- Mate:285: HeadLever:1 ↔ HeadTop:1
- Flush:111: Frame - Copy:1 ↔ ThumbScrew:1
- Mate:286: TablePt2:1 ↔ SyringeServoClamp:1
- Flush:112: TablePt2:1 ↔ SyringeServoClamp:1
- Flush:113: TablePt2:1 ↔ SyringeServoClamp:1
- Mate:287 (0.5 mm): ButtonMount:1 ↔ ButtonMountCarrier:2
- Mate:288 (0.5 mm): ButtonMount:1 ↔ ButtonMountCarrier:2
- Angle:11 (0 deg): ButtonMount:1 ↔ ButtonMountCarrier:2
- Mate:292: ButtonMountCarrier:2 ↔ ButtonLockerV2:2
- Angle:12 (0 deg): ButtonMountLegs:1 ↔ ButtonLockerV2:2
- Angle:13 (0 deg): ButtonMountCarrier:2 ↔ ButtonLockerV2:3
- Mate:295: Frame - Copy:1 ↔ BaseSyringeRackWall:1
- Mate:296: Frame - Copy:1 ↔ BaseSyringeRackWall:1
- Mate:297: SyringeBody:3 ↔ SyringEnd:4
- Flush:114: Frame - Copy:1 ↔ FrameRim:1
- Mate:298: Face:1 ↔ SensorMount:2
- Angle:14 (0 deg): HeadBottom:2 ↔ SensorMount:2
- Mate:299: Face:1 ↔ SensorMount:2
## Named parameters: d40_d20 = 0 mm, d43_d23_d10 = 0 mm, d44_d24_d11 = 0 mm, d45_d25_d12 = 0 mm, d10_d8 = 0 mm, d11_d9 = 0 mm, d12_d371 = 0 mm, d13_d372 = 0 mm, d14_d373 = 0 mm, d15_d361 = 0 mm, d16_d40_d20 = 0 mm, d17_d43_d23_d10 = 0 mm, d18_d44_d24_d11 = 0 mm, d19_d45_d25_d12 = 0 mm, d20_d8 = 0 mm, d21_d9 = 0 mm, d22_d371 = 0 mm, d23_d372 = 0 mm, d24_d373 = 0 mm, d25_d361 = 0 mm, d26_d40_d20 = 0 mm, d27_d43_d23_d10 = 0 mm, d28_d44_d24_d11 = 0 mm, d29_d45_d25_d12 = 0 mm, d30_d8 = 0 mm, d31_d9 = 0 mm, d32_d371 = 0 mm, d33_d372 = 0 mm, d34_d373 = 0 mm, d35_d361 = 0 mm, d36_d40_d20 = 0 mm, d37_d43_d23_d10 = 0 mm, d38_d44_d24_d11 = 0 mm, d39_d45_d25_d12 = 0 mm, d76_d8 = 0 mm, d77_d9 = 0 mm, d84_d81 = 0.5 mm, d85_d0 = 0 mm, d86_d1 = 0 mm, d87_d2 = 0 mm, d88_d3 = 0 mm, d89_d4 = 0 mm, d90_d5 = 0 mm, d91_d6 = 0 mm, d92_d7 = 0 mm, d93_d76_d8 = 0 mm, d94_d77_d9 = 0 mm, d95_d10 = 0 mm, d96_d11 = 0 mm, d97_d12 = 0 mm, d137_d12 = 0 mm, d140_d14 = 0 mm, d141_d15 = 0 mm, d142_d16 = 0 mm, d143_d17 = 0 mm, d144_d19 = 0 mm, d145_d20 = 0 mm, d146_d21 = 0 mm, d147_d26 = 0 mm, d148_d27 = 0 mm, d149_d28 = 0 mm, d150_d29 = 0 mm, d151_d137_d12 = 0 mm, d152_d13 = 0 mm, d153_d139 = 0.5 mm, d181_d156 = 0.25 mm, d215_d163 = 0 mm, d259_d248 = 0 mm, d260_d249 = 0 mm, d261_d250 = 0 mm, d262_d251 = 0 mm, d263_d252 = 0 mm, d264_d253 = 0 mm, d265_d254 = 0 mm, d266_d255 = 0 mm, d273_d248 = 0 mm, d274_d249 = 0 mm, d275_d250 = 0 mm, d276_d251 = 0 mm, d278_d252 = 0 mm, d279_d253 = 0 mm, d280_d254 = 0 mm, d282_d255 = 0 mm, d293_d139 = 1 mm, d379_d392_d334 = 0 mm, d380_d393_d335 = 0 mm, d387_d370 = 0 mm, d388_d374 = 0 mm, d418_d399 = 0 mm, d419_d378_d391_d333 = 0 mm
